# Autodesk Inventor assembly: Montagem_Suporte_Rolamento
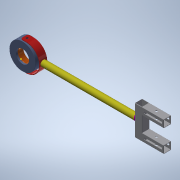
[picture p0: Inventor's stored thumbnail of the model, 180x180]
Saved by Autodesk Inventor 2022 (Build 260153000, 153)
## iProperties
Created: 2016-03-04
Part Number: Montagem_Suporte_Rolamento
Document SubType Name: Assembly
Designer: Everton
Author: Everton
## Documents named in this file (5)
- C:\Users\Alison\Documents\TCC\Peças e desenho no inventor - TCC\Peças\Montagem_Suporte_Rolamento.iam
- C:\Users\Alison\Documents\TCC\Desenhos e Montagem\desenhos e montagems inventor 15\SUPORTE_TUBO.ipt
- C:\Users\Alison\Documents\TCC\Desenhos e Montagem\desenhos e montagems inventor 15\FIXADOR_APOIO_ROLAMENTO.ipt
- C:\Users\Alison\Documents\TCC\Desenhos e Montagem\desenhos e montagems inventor 15\Apoio Tubo.ipt
- C:\Users\Alison\Documents\TCC\Desenhos e Montagem\desenhos e montagems inventor 15\MONTAGEM_ROLAMENTO.iam
## Components (4 placed, 4 different names)
1. SUPORTE_TUBO:1 — Mate:1, Flush:2, Mate:4
2. FIXADOR_APOIO_ROLAMENTO:1 — Mate:1, Mate:2, Mate:3
3. Apoio Tubo:1 — Mate:2, Mate:3, Mate:4, Mate:5
4. MONTAGEM_ROLAMENTO:1 [sub-assembly] — Mate:5
## Relationships (6: Mate 5, Flush 1)
- Mate:1: SUPORTE_TUBO:1 ↔ FIXADOR_APOIO_ROLAMENTO:1
- Flush:2: SUPORTE_TUBO:1
- Mate:2: FIXADOR_APOIO_ROLAMENTO:1 ↔ Apoio Tubo:1
- Mate:3 (85 mm): FIXADOR_APOIO_ROLAMENTO:1 ↔ Apoio Tubo:1
- Mate:4 (-695 mm): SUPORTE_TUBO:1 ↔ Apoio Tubo:1
- Mate:5: Apoio Tubo:1 ↔ MONTAGEM_ROLAMENTO:1
